# Autodesk Inventor assembly: AK-C-C39-LED-Board-Assembly2
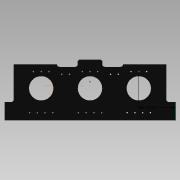
[picture p0: Inventor's stored thumbnail of the model, 180x180]
Saved by Autodesk Inventor 2016 (Build 200138000, 138)
## iProperties
Created: 2016-05-26
Part Number: AK-C-C39-LED-Board-Assembly2
Document SubType Name: Assembly
Designer: admin
Author: admin
## Documents named in this file (5)
- E:\Alex\DI-Lambda\parts\v1\AK-C-C39\AK-C-C39-LED-Board-Assembly2.iam
- E:\Alex\DI-Lambda\parts\v1\AK-C-C39\AK-C-C39-LED-Carrier-Board.ipt
- E:\Alex\DI-Lambda\parts\Common\Pin-round-2.54-female.ipt
- E:\Alex\DI-Lambda\parts\v1\AK-C-C39\AK-C-C39-LED-Module.iam
- E:\Alex\DI-Lambda\parts\Common\SSM-101-F-DH.ipt
## Components (19 placed, 4 different names)
1. AK-C-C39-LED-Carrier-Board:1 — Angle:1, Mate:30, Mate:31, Mate:32, Mate:33, Mate:34, Mate:35, Mate:36, Mate:37, Mate:38, Mate:39, Mate:46, Angle:3, Mate:49, Flush:35
2. Pin-round-2.54-female:6 — Mate:6, Flush:9, Flush:10, Mate:40, Mate:41
3. Pin-round-2.54-female:8 — Mate:6, Flush:9, Flush:10, Flush:11, Flush:12, Mate:7
4. Pin-round-2.54-female:16 — Flush:4, Flush:8, Mate:3, Mate:4
5. Pin-round-2.54-female:17 — Flush:3, Flush:4, Flush:7, Flush:8, Mate:2, Angle:1, Mate:30
6. Pin-round-2.54-female:18 — Flush:2, Flush:3, Flush:6, Flush:7, Mate:2, Mate:3
7. Pin-round-2.54-female:19 — Flush:2, Flush:6, Mate:4, Angle:2, Mate:34
8. Pin-round-2.54-female:21 — Flush:11, Flush:12, Mate:7, Angle:2, Mate:35, Mate:36, Mate:50
9. AK-C-C39-LED-Module:1 [sub-assembly] — Mate:40, Mate:41, Mate:50
10. Pin-round-2.54-female:22 — Mate:25, Mate:26, Flush:22, Flush:23, Flush:28, Flush:29
11. Pin-round-2.54-female:23 — Mate:25, Mate:27, Flush:23, Flush:24, Flush:29, Flush:30, Mate:31
12. Pin-round-2.54-female:24 — Mate:26, Flush:22, Flush:28, Mate:33
13. Pin-round-2.54-female:25 — Mate:27, Flush:24, Flush:30, Mate:32, Mate:48
14. Pin-round-2.54-female:26 — Flush:25, Mate:28, Flush:31, Mate:38, Mate:39
15. Pin-round-2.54-female:27 — Flush:25, Flush:26, Mate:28, Mate:29, Flush:31, Flush:32
16. Pin-round-2.54-female:28 — Flush:26, Mate:29, Flush:32, Mate:37, Mate:42, Mate:43
17. AK-C-C39-LED-Module:2 [sub-assembly] — Mate:42, Mate:43, Mate:48
18. SSM-101-F-DH:1 — Mate:45, Flush:34, Mate:49, Flush:36
19. SSM-101-F-DH:2 — Mate:45, Flush:34, Mate:46, Angle:3, Flush:35, Flush:36
## Relationships (55: Mate 29, Flush 23, Angle 3)
- Flush:2: Pin-round-2.54-female:18 ↔ Pin-round-2.54-female:19
- Flush:3: Pin-round-2.54-female:17 ↔ Pin-round-2.54-female:18
- Flush:4: Pin-round-2.54-female:16 ↔ Pin-round-2.54-female:17
- Flush:6: Pin-round-2.54-female:18 ↔ Pin-round-2.54-female:19
- Flush:7: Pin-round-2.54-female:17 ↔ Pin-round-2.54-female:18
- Flush:8: Pin-round-2.54-female:16 ↔ Pin-round-2.54-female:17
- Mate:2: Pin-round-2.54-female:17 ↔ Pin-round-2.54-female:18
- Mate:3: Pin-round-2.54-female:16 ↔ Pin-round-2.54-female:18
- Mate:4: Pin-round-2.54-female:16 ↔ Pin-round-2.54-female:19
- Mate:6: Pin-round-2.54-female:6 ↔ Pin-round-2.54-female:8
- Flush:9: Pin-round-2.54-female:6 ↔ Pin-round-2.54-female:8
- Flush:10: Pin-round-2.54-female:6 ↔ Pin-round-2.54-female:8
- Flush:11: Pin-round-2.54-female:8 ↔ Pin-round-2.54-female:21
- Flush:12: Pin-round-2.54-female:8 ↔ Pin-round-2.54-female:21
- Mate:7: Pin-round-2.54-female:8 ↔ Pin-round-2.54-female:21
- Angle:1 (0 deg): AK-C-C39-LED-Carrier-Board:1 ↔ Pin-round-2.54-female:17
- Angle:2 (0 deg): Pin-round-2.54-female:19 ↔ Pin-round-2.54-female:21
- Mate:25: Pin-round-2.54-female:22 ↔ Pin-round-2.54-female:23
- Mate:26: Pin-round-2.54-female:22 ↔ Pin-round-2.54-female:24
- Mate:27: Pin-round-2.54-female:23 ↔ Pin-round-2.54-female:25
- Flush:22: Pin-round-2.54-female:22 ↔ Pin-round-2.54-female:24
- Flush:23: Pin-round-2.54-female:22 ↔ Pin-round-2.54-female:23
- Flush:24: Pin-round-2.54-female:23 ↔ Pin-round-2.54-female:25
- Flush:25: Pin-round-2.54-female:26 ↔ Pin-round-2.54-female:27
- Flush:26: Pin-round-2.54-female:27 ↔ Pin-round-2.54-female:28
- Mate:28: Pin-round-2.54-female:26 ↔ Pin-round-2.54-female:27
- Mate:29: Pin-round-2.54-female:27 ↔ Pin-round-2.54-female:28
- Flush:28: Pin-round-2.54-female:22 ↔ Pin-round-2.54-female:24
- Flush:29: Pin-round-2.54-female:22 ↔ Pin-round-2.54-female:23
- Flush:30: Pin-round-2.54-female:23 ↔ Pin-round-2.54-female:25
- Mate:30: AK-C-C39-LED-Carrier-Board:1 ↔ Pin-round-2.54-female:17
- Mate:31: AK-C-C39-LED-Carrier-Board:1 ↔ Pin-round-2.54-female:23
- Mate:32: AK-C-C39-LED-Carrier-Board:1 ↔ Pin-round-2.54-female:25
- Mate:33: AK-C-C39-LED-Carrier-Board:1 ↔ Pin-round-2.54-female:24
- Mate:34: AK-C-C39-LED-Carrier-Board:1 ↔ Pin-round-2.54-female:19
- Mate:35: AK-C-C39-LED-Carrier-Board:1 ↔ Pin-round-2.54-female:21
- Mate:36: AK-C-C39-LED-Carrier-Board:1 ↔ Pin-round-2.54-female:21
- Flush:31: Pin-round-2.54-female:26 ↔ Pin-round-2.54-female:27
- Flush:32: Pin-round-2.54-female:27 ↔ Pin-round-2.54-female:28
- Mate:37: AK-C-C39-LED-Carrier-Board:1 ↔ Pin-round-2.54-female:28
- Mate:38: AK-C-C39-LED-Carrier-Board:1 ↔ Pin-round-2.54-female:26
- Mate:39: AK-C-C39-LED-Carrier-Board:1 ↔ Pin-round-2.54-female:26
- Mate:40: Pin-round-2.54-female:6 ↔ AK-C-C39-LED-Module:1
- Mate:41: Pin-round-2.54-female:6 ↔ AK-C-C39-LED-Module:1
- Mate:42: Pin-round-2.54-female:28 ↔ AK-C-C39-LED-Module:2
- Mate:43: Pin-round-2.54-female:28 ↔ AK-C-C39-LED-Module:2
- Mate:45: SSM-101-F-DH:1 ↔ SSM-101-F-DH:2
- Flush:34: SSM-101-F-DH:1 ↔ SSM-101-F-DH:2
- Mate:46: AK-C-C39-LED-Carrier-Board:1 ↔ SSM-101-F-DH:2
- Angle:3 (0 deg): AK-C-C39-LED-Carrier-Board:1 ↔ SSM-101-F-DH:2
- Mate:48: Pin-round-2.54-female:25 ↔ AK-C-C39-LED-Module:2
- Mate:49 (8 mm): AK-C-C39-LED-Carrier-Board:1 ↔ SSM-101-F-DH:1
- Flush:35 (3 mm): AK-C-C39-LED-Carrier-Board:1 ↔ SSM-101-F-DH:2
- Mate:50: Pin-round-2.54-female:21 ↔ AK-C-C39-LED-Module:1
- Flush:36: SSM-101-F-DH:1 ↔ SSM-101-F-DH:2
